# Autodesk Inventor assembly: Assembly_GaragenBox
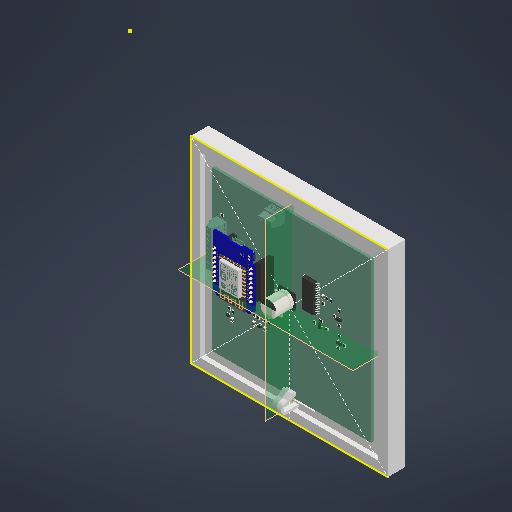
[picture p0: Inventor's stored thumbnail of the model, 512x512]
Saved by Autodesk Inventor 2027 (Build 310192000, 192)
## iProperties
Created: 2026-02-04
Part Number: Assembly_GaragenBox
Document SubType Name: Assembly
Designer: schoe
Author: schoe
## Documents named in this file (4)
- E:\GitHub\garage-project\pcb\Garage-Box-Project\Assembly_GaragenBox.iam
- E:\GitHub\garage-project\pcb\Garage-Box-Project\Box_with_PCBRefernce.ipt
- E:\GitHub\garage-project\pcb\Garage-Box-Project\Clipper.ipt
- E:\GitHub\garage-project\pcb\Garage-Box-Project\SolidBody_PCB_better.ipt
## Components (3 placed, 3 different names)
1. Box_with_PCBRefernce:1 — Mate:1, Flush:11, Flush:10, Mate:2, Mate:3, Flush:12, Flush:13
2. Clipper:1 — Mate:1, Flush:11, Flush:10
3. SolidBody_PCB_better:1 — Mate:2, Mate:3, Flush:12, Flush:13
## Relationships (7: Flush 4, Mate 3)
- Mate:1: Box_with_PCBRefernce:1 ↔ Clipper:1
- Flush:11: Box_with_PCBRefernce:1 ↔ Clipper:1
- Flush:10: Box_with_PCBRefernce:1 ↔ Clipper:1
- Mate:2: Box_with_PCBRefernce:1 ↔ SolidBody_PCB_better:1
- Mate:3: Box_with_PCBRefernce:1 ↔ SolidBody_PCB_better:1
- Flush:12: Box_with_PCBRefernce:1 ↔ SolidBody_PCB_better:1
- Flush:13: Box_with_PCBRefernce:1 ↔ SolidBody_PCB_better:1
